# Autodesk Inventor assembly: prostkatna waska wysoka lacznik
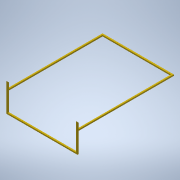
[picture p0: Inventor's stored thumbnail of the model, 180x180]
Saved by Autodesk Inventor 2021 (Build 250183000, 183)
## iProperties
Created: 2024-04-18
Part Number: prostkatna waska wysoka lacznik
Document SubType Name: Assembly
Designer: Michal
Author: Michal
## Documents named in this file (7)
- C:\Users\Michal\Documents\GitHub\PNW_PhotoBoothFrame_3D\prostkatna waska wysoka lacznik.iam
- C:\Users\Michal\Documents\GitHub\PNW_PhotoBoothFrame_3D\Gora L1500.ipt
- C:\Users\Michal\Documents\GitHub\PNW_PhotoBoothFrame_3D\Noga L L2000.ipt
- C:\Users\Michal\Documents\GitHub\PNW_PhotoBoothFrame_3D\Noga P L2000.ipt
- C:\Users\Michal\Documents\GitHub\PNW_PhotoBoothFrame_3D\Naroznik.iam
- C:\Users\Michal\Documents\GitHub\PNW_PhotoBoothFrame_3D\Stopa v2 P.iam
- C:\Users\Michal\Documents\GitHub\PNW_PhotoBoothFrame_3D\Stopa v2 L.iam
## Components (10 placed, 6 different names)
1. Stopa v2 L:1 [sub-assembly] — Mate:1, Flush:3, Mate:2, Flush:8, Flush:12, Flush:13
2. Stopa v2 P:1 [sub-assembly] — Mate:10, Flush:4, Flush:5, Mate:11, Flush:8
3. Naroznik:1 [sub-assembly] — Mate:12, Mate:13, Mate:14, Mate:15
4. Naroznik:2 [sub-assembly] — Mate:7, Mate:8, Mate:9, Mate:17, Mate:40
5. Noga L L2000:1 — Mate:1, Flush:3, Mate:2, Mate:7, Mate:8, Mate:9
6. Noga P L2000:1 — Mate:10, Flush:4, Flush:5, Mate:11, Mate:12, Mate:13, Mate:14, Flush:6
7. Gora L1500:1 — Flush:6, Mate:15, Mate:17, Mate:38, Flush:7, Mate:39, Mate:40
8. Naroznik:3 [sub-assembly] — Mate:58, Flush:12, Flush:13
9. Naroznik:4 [sub-assembly]
10. Gora L1500:2 — Mate:58
## Relationships (27: Mate 19, Flush 8)
- Mate:1: Stopa v2 L:1 ↔ Noga L L2000:1
- Flush:3: Stopa v2 L:1 ↔ Noga L L2000:1
- Mate:2: Stopa v2 L:1 ↔ Noga L L2000:1
- Mate:7: Naroznik:2 ↔ Noga L L2000:1
- Mate:8: Naroznik:2 ↔ Noga L L2000:1
- Mate:9: Naroznik:2 ↔ Noga L L2000:1
- Mate:10: Stopa v2 P:1 ↔ Noga P L2000:1
- Flush:4: Stopa v2 P:1 ↔ Noga P L2000:1
- Flush:5: Stopa v2 P:1 ↔ Noga P L2000:1
- Mate:11: Stopa v2 P:1 ↔ Noga P L2000:1
- Mate:12: Naroznik:1 ↔ Noga P L2000:1
- Mate:13: Naroznik:1 ↔ Noga P L2000:1
- Mate:14: Naroznik:1 ↔ Noga P L2000:1
- Flush:6: Noga P L2000:1 ↔ Gora L1500:1
- Mate:15: Naroznik:1 ↔ Gora L1500:1
- Mate:17: Naroznik:2 ↔ Gora L1500:1
- Mate:38: Gora L1500:1
- Flush:7: Gora L1500:1
- Mate:39: Gora L1500:1
- Flush:8: Stopa v2 L:1 ↔ Stopa v2 P:1
- Mate:40: Naroznik:2 ↔ Gora L1500:1
- [Mate]: Naroznik:3 ↔ Gora L1500:2
- [Mate]: Naroznik:4 ↔ Gora L1500:2
- [Mate]: Naroznik:4 ↔ Gora L1500:2
- Mate:58: Naroznik:3 ↔ Gora L1500:2
- Flush:12: Stopa v2 L:1 ↔ Naroznik:3
- Flush:13: Stopa v2 L:1 ↔ Naroznik:3
## Named parameters: d55_d50 = 0 mm, d56_d21 = 0 mm, d57_d23 = 0 mm
